# Autodesk Inventor assembly: dron
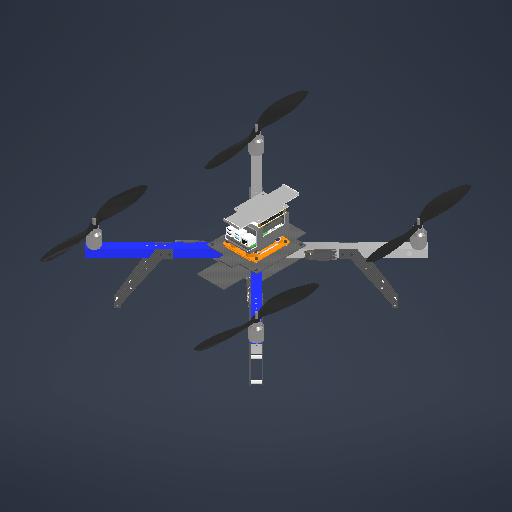
[picture p0: Inventor's stored thumbnail of the model, 512x512]
Saved by Autodesk Inventor 2026.2 (Build 302298000, 298)
## iProperties
Created: 2025-09-23
Part Number: dron
Document SubType Name: Assembly
Designer: rodri
Mass: 1213.65 g
Surface Area: 5864.79 cm^2
Volume: 390.414 cm^3
Density: 3.10863 g/cm^3
Author: rodri
## Documents named in this file (18)
- D:\Documentos\inventor\Dron\dron.iam
- D:\Documentos\inventor\Dron\swtc2.ipt
- D:\Documentos\inventor\Dron\brazo.ipt
- D:\Documentos\inventor\Dron\motor.ipt
- D:\Documentos\inventor\Dron\Ensa_carcasa.iam
- D:\Documentos\inventor\Dron\swtc1.ipt
- D:\Documentos\inventor\Dron\pata.ipt
- D:\Documentos\inventor\Dron\GEMFAN 11x4.7.ipt
- C:\Users\rodri\Documents\Inventor\Content Center Files\R2026\es-ES\ISO 7045  H\ISO 7045 - M3 x 25_ - 4.8 - H - ISO.ipt
- C:\Users\rodri\Documents\Inventor\Content Center Files\R2026\es-ES\ISO 4036(2)\ISO 4036 - M3(2).ipt
- C:\Users\rodri\Documents\Inventor\Content Center Files\R2026\es-ES\ISO 4035(2)\ISO 4035 - M3 - ISO.ipt
- C:\Users\rodri\Documents\Inventor\Content Center Files\R2026\es-ES\ISO 7045  H\ISO 7045 - M3 x 30_ - 4.8 - H - ISO.ipt
- D:\Documentos\inventor\Dron\pataUnion.ipt
- D:\Documentos\inventor\Dron\NAVIO2.ipt
- D:\Documentos\inventor\Dron\ESC.ipt
- D:\Documentos\inventor\Dron\posteNAVIO.ipt
- D:\Documentos\inventor\Dron\Soporte_bateria_p1.ipt
- D:\Documentos\inventor\Dron\relleno.ipt
## Components (78 placed, 17 different names)
1. swtc2:1 — Coincidencia:1, Coincidencia:3, Coincidencia:5, Coincidencia:6, Coincidencia:7, Coincidencia:8, Coincidencia:9, Coincidencia:10, Coincidencia:15, Coincidencia:106, Coincidencia:108, Coincidencia:110, Coincidencia:112
2. brazo:1 — Coincidencia:1, Coincidencia:9, Coincidencia:13, Coincidencia:29, Coincidencia:31, Coincidencia:35, Coincidencia:36, Coincidencia:141
3. brazo:2 — Coincidencia:3, Coincidencia:10, Coincidencia:12, Coincidencia:25, Coincidencia:27, Coincidencia:33, Coincidencia:34, Coincidencia:138
4. brazo:3 — Coincidencia:7, Coincidencia:8, Coincidencia:14, Coincidencia:16, Coincidencia:17, Coincidencia:18, Coincidencia:19, Coincidencia:20, Coincidencia:140
5. brazo:4 — Coincidencia:5, Coincidencia:6, Coincidencia:11, Coincidencia:21, Coincidencia:23, Coincidencia:24, Coincidencia:32, Coincidencia:139
6. motor:1 — Coincidencia:11, Coincidencia:41, Coincidencia:43
7. motor:2 — Coincidencia:12, Coincidencia:40, Coincidencia:44
8. motor:3 — Coincidencia:13, Coincidencia:39, Coincidencia:42
9. motor:4 — Coincidencia:14, Coincidencia:37, Coincidencia:38
10. Ensa_carcasa:1 [sub-assembly] — Coincidencia:15, Coincidencia:90, Coincidencia:92, Coincidencia:94, Coincidencia:96, Coincidencia:137
11. swtc1:1 — Coincidencia:16, Coincidencia:81, Coincidencia:82, Coincidencia:83, Coincidencia:84, Coincidencia:85, Coincidencia:86, Coincidencia:87, Coincidencia:88, Coincidencia:89, Coincidencia:91, Coincidencia:93, Coincidencia:95, Coincidencia:97, Coincidencia:98, Coincidencia:99, Coincidencia:100, Coincidencia:101, Coincidencia:102, Coincidencia:103, Coincidencia:104, Coincidencia:105, Coincidencia:107, Coincidencia:109, Coincidencia:111, Coincidencia:147
12. pata:1 — Coincidencia:23, Coincidencia:24, Coincidencia:49, Coincidencia:50, Coincidencia:51, Coincidencia:52, Coincidencia:53, Coincidencia:55, Coincidencia:126, Coincidencia:128, Coincidencia:130
13. pata:2 — Coincidencia:21, Coincidencia:32, Coincidencia:54, Coincidencia:56, Coincidencia:125, Coincidencia:127, Coincidencia:129
14. pata:3 — Coincidencia:17, Coincidencia:18, Coincidencia:57, Coincidencia:58, Coincidencia:59, Coincidencia:60, Coincidencia:61, Coincidencia:63, Coincidencia:119, Coincidencia:121, Coincidencia:123
15. pata:4 — Coincidencia:19, Coincidencia:20, Coincidencia:62, Coincidencia:64, Coincidencia:120, Coincidencia:122, Coincidencia:124
16. pata:5 — Coincidencia:27, Coincidencia:33, Coincidencia:78, Coincidencia:80, Coincidencia:132, Coincidencia:134, Coincidencia:136
17. pata:6 — Coincidencia:25, Coincidencia:34, Coincidencia:73, Coincidencia:74, Coincidencia:75, Coincidencia:76, Coincidencia:77, Coincidencia:79, Coincidencia:131, Coincidencia:133, Coincidencia:135
18. pata:7 — Coincidencia:29, Coincidencia:35, Coincidencia:70, Coincidencia:72, Coincidencia:113, Coincidencia:116, Coincidencia:118
19. pata:8 — Coincidencia:31, Coincidencia:36, Coincidencia:65, Coincidencia:66, Coincidencia:67, Coincidencia:68, Coincidencia:69, Coincidencia:71, Coincidencia:114, Coincidencia:115, Coincidencia:117
20. GEMFAN 11x4.7:1 — Coincidencia:37, Coincidencia:38
21. GEMFAN 11x4.7:2 — Coincidencia:39, Coincidencia:42
22. GEMFAN 11x4.7:3 — Coincidencia:40, Coincidencia:44
23. GEMFAN 11x4.7:4 — Coincidencia:41, Coincidencia:43
24. ISO 7045 H M3 x 25 - 4.8 - H:2 — Coincidencia:49, Coincidencia:50
25. ISO 4035 M3:1 — Coincidencia:53, Coincidencia:54
26. ISO 7045 H M3 x 25 - 4.8 - H:3 — Coincidencia:51, Coincidencia:52
27. ISO 4035 M3:2 — Coincidencia:55, Coincidencia:56
28. ISO 7045 H M3 x 25 - 4.8 - H:4 — Coincidencia:57, Coincidencia:58
29. ISO 4036 M3:1 — Coincidencia:61, Coincidencia:62
30. ISO 7045 H M3 x 25 - 4.8 - H:5 — Coincidencia:59, Coincidencia:60
31. ISO 4036 M3:2 — Coincidencia:63, Coincidencia:64
32. ISO 7045 H M3 x 25 - 4.8 - H:6 — Coincidencia:65, Coincidencia:66
33. ISO 4036 M3:3 — Coincidencia:69, Coincidencia:70
34. ISO 7045 H M3 x 25 - 4.8 - H:7 — Coincidencia:67, Coincidencia:68
35. ISO 4036 M3:4 — Coincidencia:71, Coincidencia:72
36. ISO 7045 H M3 x 25 - 4.8 - H:8 — Coincidencia:73, Coincidencia:74
37. ISO 4036 M3:5 — Coincidencia:77, Coincidencia:78
38. ISO 7045 H M3 x 25 - 4.8 - H:9 — Coincidencia:75, Coincidencia:76
39. ISO 4036 M3:6 — Coincidencia:79, Coincidencia:80
40. ISO 7045 H M3 x 30 - 4.8 - H:1 — Coincidencia:81, Coincidencia:82
41. ISO 4036 M3:7 — Coincidencia:89, Coincidencia:90
42. ISO 7045 H M3 x 30 - 4.8 - H:2 — Coincidencia:83, Coincidencia:84
43. ISO 7045 H M3 x 30 - 4.8 - H:3 — Coincidencia:85, Coincidencia:86
44. ISO 7045 H M3 x 30 - 4.8 - H:4 — Coincidencia:87, Coincidencia:88
45. ISO 4036 M3:8 — Coincidencia:91, Coincidencia:92
46. ISO 4036 M3:9 — Coincidencia:93, Coincidencia:94
47. ISO 4036 M3:10 — Coincidencia:95, Coincidencia:96
48. ISO 7045 H M3 x 25 - 4.8 - H:10 — Coincidencia:97, Coincidencia:98
49. ISO 4036 M3:11 — Coincidencia:105, Coincidencia:106
50. ISO 7045 H M3 x 25 - 4.8 - H:11 — Coincidencia:99, Coincidencia:100
51. ISO 7045 H M3 x 25 - 4.8 - H:12 — Coincidencia:101, Coincidencia:102
52. ISO 7045 H M3 x 25 - 4.8 - H:13 — Coincidencia:103, Coincidencia:104
53. ISO 4036 M3:12 — Coincidencia:107, Coincidencia:108
54. ISO 4036 M3:13 — Coincidencia:109, Coincidencia:110
55. ISO 4036 M3:14 — Coincidencia:111, Coincidencia:112
56. pataUnion:1 — Coincidencia:117, Coincidencia:118
57. pataUnion:2 — Coincidencia:115, Coincidencia:116
58. pataUnion:3 — Coincidencia:113, Coincidencia:114
59. pataUnion:4 — Coincidencia:123, Coincidencia:124
60. pataUnion:5 — Coincidencia:121, Coincidencia:122
61. pataUnion:6 — Coincidencia:119, Coincidencia:120
62. pataUnion:7 — Coincidencia:129, Coincidencia:130
63. pataUnion:8 — Coincidencia:127, Coincidencia:128
64. pataUnion:9 — Coincidencia:125, Coincidencia:126
65. pataUnion:10 — Coincidencia:135, Coincidencia:136
66. pataUnion:11 — Coincidencia:133, Coincidencia:134
67. pataUnion:12 — Coincidencia:131, Coincidencia:132
68. NAVIO2:1 — Coincidencia:137, Coincidencia:142, Coincidencia:143, Coincidencia:144, Coincidencia:145
69. ESC:1 — Coincidencia:138
70. ESC:2 — Coincidencia:139
71. ESC:3 — Coincidencia:140
72. ESC:4 — Coincidencia:141
73. posteNAVIO:1 — Coincidencia:144
74. posteNAVIO:2 — Coincidencia:142
75. posteNAVIO:3 — Coincidencia:145
76. posteNAVIO:4 — Coincidencia:143, Coincidencia:146
77. Soporte_bateria_p1:1 — Coincidencia:146
78. relleno:1 — Coincidencia:147
## Relationships (137: Mate 137)
- Coincidencia:1 [Mate]: swtc2:1 ↔ brazo:1
- Coincidencia:3 [Mate]: swtc2:1 ↔ brazo:2
- Coincidencia:5 [Mate]: swtc2:1 ↔ brazo:4
- Coincidencia:6 [Mate]: swtc2:1 ↔ brazo:4
- Coincidencia:7 [Mate]: swtc2:1 ↔ brazo:3
- Coincidencia:8 [Mate]: swtc2:1 ↔ brazo:3
- Coincidencia:9 [Mate]: swtc2:1 ↔ brazo:1
- Coincidencia:10 [Mate]: swtc2:1 ↔ brazo:2
- Coincidencia:11 [Mate]: brazo:4 ↔ motor:1
- Coincidencia:12 [Mate]: brazo:2 ↔ motor:2
- Coincidencia:13 [Mate]: brazo:1 ↔ motor:3
- Coincidencia:14 [Mate]: brazo:3 ↔ motor:4
- Coincidencia:15 [Mate]: swtc2:1 ↔ Ensa_carcasa:1
- Coincidencia:16 [Mate]: brazo:3 ↔ swtc1:1
- Coincidencia:17 [Mate]: brazo:3 ↔ pata:3
- Coincidencia:18 [Mate]: brazo:3 ↔ pata:3
- Coincidencia:19 [Mate]: brazo:3 ↔ pata:4
- Coincidencia:20 [Mate]: brazo:3 ↔ pata:4
- Coincidencia:21 [Mate]: brazo:4 ↔ pata:2
- Coincidencia:23 [Mate]: brazo:4 ↔ pata:1
- Coincidencia:24 [Mate]: brazo:4 ↔ pata:1
- Coincidencia:25 [Mate]: brazo:2 ↔ pata:6
- Coincidencia:27 [Mate]: brazo:2 ↔ pata:5
- Coincidencia:29 [Mate]: brazo:1 ↔ pata:7
- Coincidencia:31 [Mate]: brazo:1 ↔ pata:8
- Coincidencia:32 [Mate]: brazo:4 ↔ pata:2
- Coincidencia:33 [Mate]: brazo:2 ↔ pata:5
- Coincidencia:34 [Mate]: brazo:2 ↔ pata:6
- Coincidencia:35 [Mate]: brazo:1 ↔ pata:7
- Coincidencia:36 [Mate]: brazo:1 ↔ pata:8
- Coincidencia:37 [Mate]: motor:4 ↔ GEMFAN 11x4.7:1
- Coincidencia:38 [Mate]: motor:4 ↔ GEMFAN 11x4.7:1
- Coincidencia:39 [Mate]: motor:3 ↔ GEMFAN 11x4.7:2
- Coincidencia:40 [Mate]: motor:2 ↔ GEMFAN 11x4.7:3
- Coincidencia:41 [Mate]: motor:1 ↔ GEMFAN 11x4.7:4
- Coincidencia:42 [Mate]: motor:3 ↔ GEMFAN 11x4.7:2
- Coincidencia:43 [Mate]: motor:1 ↔ GEMFAN 11x4.7:4
- Coincidencia:44 [Mate]: motor:2 ↔ GEMFAN 11x4.7:3
- Coincidencia:49 [Mate]: pata:1 ↔ ISO 7045 H M3 x 25 - 4.8 - H:2
- Coincidencia:50 [Mate]: pata:1 ↔ ISO 7045 H M3 x 25 - 4.8 - H:2
- Coincidencia:51 [Mate]: pata:1 ↔ ISO 7045 H M3 x 25 - 4.8 - H:3
- Coincidencia:52 [Mate]: pata:1 ↔ ISO 7045 H M3 x 25 - 4.8 - H:3
- Coincidencia:53 [Mate]: pata:1 ↔ ISO 4035 M3:1
- Coincidencia:54 [Mate]: pata:2 ↔ ISO 4035 M3:1
- Coincidencia:55 [Mate]: pata:1 ↔ ISO 4035 M3:2
- Coincidencia:56 [Mate]: pata:2 ↔ ISO 4035 M3:2
- Coincidencia:57 [Mate]: pata:3 ↔ ISO 7045 H M3 x 25 - 4.8 - H:4
- Coincidencia:58 [Mate]: pata:3 ↔ ISO 7045 H M3 x 25 - 4.8 - H:4
- Coincidencia:59 [Mate]: pata:3 ↔ ISO 7045 H M3 x 25 - 4.8 - H:5
- Coincidencia:60 [Mate]: pata:3 ↔ ISO 7045 H M3 x 25 - 4.8 - H:5
- Coincidencia:61 [Mate]: pata:3 ↔ ISO 4036 M3:1
- Coincidencia:62 [Mate]: pata:4 ↔ ISO 4036 M3:1
- Coincidencia:63 [Mate]: pata:3 ↔ ISO 4036 M3:2
- Coincidencia:64 [Mate]: pata:4 ↔ ISO 4036 M3:2
- Coincidencia:65 [Mate]: pata:8 ↔ ISO 7045 H M3 x 25 - 4.8 - H:6
- Coincidencia:66 [Mate]: pata:8 ↔ ISO 7045 H M3 x 25 - 4.8 - H:6
- Coincidencia:67 [Mate]: pata:8 ↔ ISO 7045 H M3 x 25 - 4.8 - H:7
- Coincidencia:68 [Mate]: pata:8 ↔ ISO 7045 H M3 x 25 - 4.8 - H:7
- Coincidencia:69 [Mate]: pata:8 ↔ ISO 4036 M3:3
- Coincidencia:70 [Mate]: pata:7 ↔ ISO 4036 M3:3
- Coincidencia:71 [Mate]: pata:8 ↔ ISO 4036 M3:4
- Coincidencia:72 [Mate]: pata:7 ↔ ISO 4036 M3:4
- Coincidencia:73 [Mate]: pata:6 ↔ ISO 7045 H M3 x 25 - 4.8 - H:8
- Coincidencia:74 [Mate]: pata:6 ↔ ISO 7045 H M3 x 25 - 4.8 - H:8
- Coincidencia:75 [Mate]: pata:6 ↔ ISO 7045 H M3 x 25 - 4.8 - H:9
- Coincidencia:76 [Mate]: pata:6 ↔ ISO 7045 H M3 x 25 - 4.8 - H:9
- Coincidencia:77 [Mate]: pata:6 ↔ ISO 4036 M3:5
- Coincidencia:78 [Mate]: pata:5 ↔ ISO 4036 M3:5
- Coincidencia:79 [Mate]: pata:6 ↔ ISO 4036 M3:6
- Coincidencia:80 [Mate]: pata:5 ↔ ISO 4036 M3:6
- Coincidencia:81 [Mate]: swtc1:1 ↔ ISO 7045 H M3 x 30 - 4.8 - H:1
- Coincidencia:82 [Mate]: swtc1:1 ↔ ISO 7045 H M3 x 30 - 4.8 - H:1
- Coincidencia:83 [Mate]: swtc1:1 ↔ ISO 7045 H M3 x 30 - 4.8 - H:2
- Coincidencia:84 [Mate]: swtc1:1 ↔ ISO 7045 H M3 x 30 - 4.8 - H:2
- Coincidencia:85 [Mate]: swtc1:1 ↔ ISO 7045 H M3 x 30 - 4.8 - H:3
- Coincidencia:86 [Mate]: swtc1:1 ↔ ISO 7045 H M3 x 30 - 4.8 - H:3
- Coincidencia:87 [Mate]: swtc1:1 ↔ ISO 7045 H M3 x 30 - 4.8 - H:4
- Coincidencia:88 [Mate]: swtc1:1 ↔ ISO 7045 H M3 x 30 - 4.8 - H:4
- Coincidencia:89 [Mate]: swtc1:1 ↔ ISO 4036 M3:7
- Coincidencia:90 [Mate]: Ensa_carcasa:1 ↔ ISO 4036 M3:7
- Coincidencia:91 [Mate]: swtc1:1 ↔ ISO 4036 M3:8
- Coincidencia:92 [Mate]: Ensa_carcasa:1 ↔ ISO 4036 M3:8
- Coincidencia:93 [Mate]: swtc1:1 ↔ ISO 4036 M3:9
- Coincidencia:94 [Mate]: Ensa_carcasa:1 ↔ ISO 4036 M3:9
- Coincidencia:95 [Mate]: swtc1:1 ↔ ISO 4036 M3:10
- Coincidencia:96 [Mate]: Ensa_carcasa:1 ↔ ISO 4036 M3:10
- Coincidencia:97 [Mate]: swtc1:1 ↔ ISO 7045 H M3 x 25 - 4.8 - H:10
- Coincidencia:98 [Mate]: swtc1:1 ↔ ISO 7045 H M3 x 25 - 4.8 - H:10
- Coincidencia:99 [Mate]: swtc1:1 ↔ ISO 7045 H M3 x 25 - 4.8 - H:11
- Coincidencia:100 [Mate]: swtc1:1 ↔ ISO 7045 H M3 x 25 - 4.8 - H:11
- Coincidencia:101 [Mate]: swtc1:1 ↔ ISO 7045 H M3 x 25 - 4.8 - H:12
- Coincidencia:102 [Mate]: swtc1:1 ↔ ISO 7045 H M3 x 25 - 4.8 - H:12
- Coincidencia:103 [Mate]: swtc1:1 ↔ ISO 7045 H M3 x 25 - 4.8 - H:13
- Coincidencia:104 [Mate]: swtc1:1 ↔ ISO 7045 H M3 x 25 - 4.8 - H:13
- Coincidencia:105 [Mate]: swtc1:1 ↔ ISO 4036 M3:11
- Coincidencia:106 [Mate]: swtc2:1 ↔ ISO 4036 M3:11
- Coincidencia:107 [Mate]: swtc1:1 ↔ ISO 4036 M3:12
- Coincidencia:108 [Mate]: swtc2:1 ↔ ISO 4036 M3:12
- Coincidencia:109 [Mate]: swtc1:1 ↔ ISO 4036 M3:13
- Coincidencia:110 [Mate]: swtc2:1 ↔ ISO 4036 M3:13
- Coincidencia:111 [Mate]: swtc1:1 ↔ ISO 4036 M3:14
- Coincidencia:112 [Mate]: swtc2:1 ↔ ISO 4036 M3:14
- Coincidencia:113 [Mate]: pata:7 ↔ pataUnion:3
- Coincidencia:114 [Mate]: pata:8 ↔ pataUnion:3
- Coincidencia:115 [Mate]: pata:8 ↔ pataUnion:2
- Coincidencia:116 [Mate]: pata:7 ↔ pataUnion:2
- Coincidencia:117 [Mate]: pata:8 ↔ pataUnion:1
- Coincidencia:118 [Mate]: pata:7 ↔ pataUnion:1
- Coincidencia:119 [Mate]: pata:3 ↔ pataUnion:6
- Coincidencia:120 [Mate]: pata:4 ↔ pataUnion:6
- Coincidencia:121 [Mate]: pata:3 ↔ pataUnion:5
- Coincidencia:122 [Mate]: pata:4 ↔ pataUnion:5
- Coincidencia:123 [Mate]: pata:3 ↔ pataUnion:4
- Coincidencia:124 [Mate]: pata:4 ↔ pataUnion:4
- Coincidencia:125 [Mate]: pata:2 ↔ pataUnion:9
- Coincidencia:126 [Mate]: pata:1 ↔ pataUnion:9
- Coincidencia:127 [Mate]: pata:2 ↔ pataUnion:8
- Coincidencia:128 [Mate]: pata:1 ↔ pataUnion:8
- Coincidencia:129 [Mate]: pata:2 ↔ pataUnion:7
- Coincidencia:130 [Mate]: pata:1 ↔ pataUnion:7
- Coincidencia:131 [Mate]: pata:6 ↔ pataUnion:12
- Coincidencia:132 [Mate]: pata:5 ↔ pataUnion:12
- Coincidencia:133 [Mate]: pata:6 ↔ pataUnion:11
- Coincidencia:134 [Mate]: pata:5 ↔ pataUnion:11
- Coincidencia:135 [Mate]: pata:6 ↔ pataUnion:10
- Coincidencia:136 [Mate]: pata:5 ↔ pataUnion:10
- Coincidencia:137 [Mate]: Ensa_carcasa:1 ↔ NAVIO2:1
- Coincidencia:138 [Mate]: brazo:2 ↔ ESC:1
- Coincidencia:139 [Mate]: brazo:4 ↔ ESC:2
- Coincidencia:140 [Mate]: brazo:3 ↔ ESC:3
- Coincidencia:141 [Mate]: brazo:1 ↔ ESC:4
- Coincidencia:142 [Mate]: NAVIO2:1 ↔ posteNAVIO:2
- Coincidencia:143 [Mate]: NAVIO2:1 ↔ posteNAVIO:4
- Coincidencia:144 [Mate]: NAVIO2:1 ↔ posteNAVIO:1
- Coincidencia:145 [Mate]: NAVIO2:1 ↔ posteNAVIO:3
- Coincidencia:146 [Mate]: posteNAVIO:4 ↔ Soporte_bateria_p1:1
- Coincidencia:147 [Mate]: swtc1:1 ↔ relleno:1
## Named parameters: Finish1_Area = 360.31, Finish1_Thickness = 0.05 mm, Finish2_Area = 213.398, Finish2_Thickness = 0.05 mm, Finish3_Area = 50.1031, Finish3_Thickness = 0.05 mm, Finish4_Area = 140.396, Finish4_Thickness = 0.05 mm
note: some values were not read from the file. Shown as the stored number, unit unknown: "Finish1_Area", "Finish2_Area", "Finish3_Area", "Finish4_Area".
